# Autodesk Inventor assembly: Zespół1
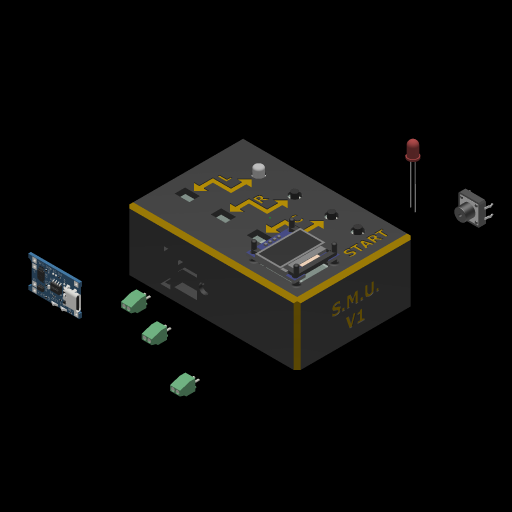
[picture p0: Inventor's stored thumbnail of the model, 512x512]
Saved by Autodesk Inventor 2024.4 (Build 284460000, 460)
## iProperties
Created: 2026-01-14
Part Number: Zespół1
Document SubType Name: Assembly
Designer: User
Author: User
## iProperties of the stored document 5mm_LED_Red.ipt
Created: 2026-01-16
Part Number: 5mm_LED_Red
Material: Generic
Document SubType Name: Modeling
Designer: rk
Mass: 0.169759 g
Surface Area: 2.48677 cm^2
Volume: 0.169759 cm^3
Density: 1 g/cm^3
Appearance: Domyślna
Author: rk
Revision Number: 0
Sending System: Autodesk Inventor 2025
## Documents named in this file (13)
- **C:\Users\Duszy\Desktop\Projekty\S.M.T\Obudowa\Zespół1.iam*LocalDocs*xAaaaa5caAaaaaaaaAaaaq10vPe*5mm_LED_Red.ipt
- C:\Users\Duszy\Desktop\Projekty\S.M.T\Obudowa\Zespół1.iam
- C:\Users\Duszy\Downloads\raspberry-pi-pico-w-2.snapshot.8\Raspberry_Pi_Pico_W.ipt
- C:\Users\Duszy\Desktop\Projekty\S.M.T\Miernik\Miernik.ipt
- C:\Users\Duszy\Desktop\Projekty\S.M.T\Obudowa\spod.ipt
- C:\Users\Duszy\Desktop\Projekty\S.M.T\Obudowa\atrapa_ogniwa.ipt
- C:\Users\Duszy\Desktop\Projekty\S.M.T\Obudowa\gora.ipt
- C:\Users\Duszy\Downloads\0-9-inch-i2c-oled-128x64-display-module-1.snapshot.1\0.9 inch I2C OLED 128×64 Display Module_jhalak.ipt
- C:\Users\Duszy\Desktop\Projekty\S.M.T\Obudowa\button.ipt
- C:\Users\Duszy\Desktop\Projekty\S.M.T\Obudowa\TerminalBlock_Phoenix_MPT-0,5-2-2.54_1x02_P2.54mm_Horizontal\TerminalBlock_Phoenix_MPT-0,5-2-2.54_1x02_P2.54mm_Horizontal\TerminalBlock_Phoenix_MPT-0,5-2-2.54_1x02_.ipt
- C:\Users\Duszy\Desktop\Projekty\S.M.T\Obudowa\TP4056_Charging_Module_Type_C\TP4056_Charging_Module_Type_C\TP4056_Charging_Module_Type_C.ipt
- C:\Users\Duszy\Desktop\Projekty\S.M.T\Obudowa\12x12x8mm\12x12x8mm\12x12x8mm.ipt
- C:\Users\Duszy\Desktop\Projekty\S.M.T\Obudowa\5mm_LED_Red.ipt
## Components (13 placed, 11 different names)
1. Miernik:1 — Obrotowe:2
2. spod:1 — Obrotowe:1, Obrotowe:2, Sztywne:4
3. Raspberry_Pi_Pico_W:1 — Obrotowe:1
4. atrapa_ogniwa:1
5. gora:1 — Sztywne:4, Sztywne:5
6. 0.9 inch I2C OLED 128×64 Display Module_jhalak:1
7. button:2 — Sztywne:5
8. TerminalBlock_Phoenix_MPT-0,5-2-2.54_1x02_:1
9. TerminalBlock_Phoenix_MPT-0,5-2-2.54_1x02_:2
10. TerminalBlock_Phoenix_MPT-0,5-2-2.54_1x02_:3
11. 5mm_LED_Red:1
12. TP4056_Charging_Module_Type_C:1
13. 12x12x8mm:1
## Relationships (4: RevoluteJoint 2, WeldJoint 2)
- Obrotowe:1 [RevoluteJoint] (-5 mm): spod:1 ↔ Raspberry_Pi_Pico_W:1
- Obrotowe:2 [RevoluteJoint] (-1 mm): Miernik:1 ↔ spod:1
- Sztywne:4 [WeldJoint] (1 mm): spod:1 ↔ gora:1
- Sztywne:5 [WeldJoint]: gora:1 ↔ button:2
